# Autodesk Inventor assembly: Y-idler
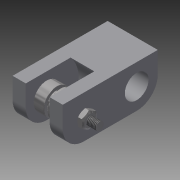
[picture p0: Inventor's stored thumbnail of the model, 180x180]
Saved by Autodesk Inventor 2015 (Build 190159000, 159)
## iProperties
Created: 2015-04-28
Part Number: Y-idler
Document SubType Name: Assembly
Designer: X
Author: X
## Documents named in this file (5)
- G:\3d printer\Prusa_i3\CAD\Y-idler.iam
- G:\3d printer\Prusa_i3\CAD\3d_printer_part\Y-idler.ipt
- G:\3d printer\Prusa_i3\CAD\standard_parts\DIN 625 SKF(4)\DIN 625 SKF - SKF 623-2Z.ipt
- G:\3d printer\Prusa_i3\CAD\standard_parts\ANSI B18.6.7M(00)\ANSI B18.6.7M - M3x0.5 x 25(4).ipt
- G:\3d printer\Prusa_i3\CAD\standard_parts\DIN 934\DIN 934 - M3 x 0.5.ipt
## Components (5 placed, 4 different names)
1. Y-idler:1 — Insert:1, Insert:2, Cylindrical:1, Mate:1, Mate:2
2. DIN 625 SKF- with two Z shields SKF 623-2Z:1 — Insert:1
3. DIN 625 SKF- with two Z shields SKF 623-2Z:2 — Insert:2
4. Cross Recessed Pan Head Machine Screw - Type I - Metric M3x0.5 x 25:1 — Cylindrical:1, Mate:1, Cylindrical:2
5. DIN 934 - replaced by DIN EN 24032/28673/28674 M3:1 — Cylindrical:2, Mate:2
## Relationships (6: Insert 2, CylindricalJoint 2, Mate 2)
- Insert:1: Y-idler:1 ↔ DIN 625 SKF- with two Z shields SKF 623-2Z:1
- Insert:2: Y-idler:1 ↔ DIN 625 SKF- with two Z shields SKF 623-2Z:2
- Cylindrical:1: Y-idler:1 ↔ Cross Recessed Pan Head Machine Screw - Type I - Metric M3x0.5 x 25:1
- Mate:1: Y-idler:1 ↔ Cross Recessed Pan Head Machine Screw - Type I - Metric M3x0.5 x 25:1
- Cylindrical:2: Cross Recessed Pan Head Machine Screw - Type I - Metric M3x0.5 x 25:1 ↔ DIN 934 - replaced by DIN EN 24032/28673/28674 M3:1
- Mate:2: Y-idler:1 ↔ DIN 934 - replaced by DIN EN 24032/28673/28674 M3:1
